# Autodesk Inventor assembly: Femto
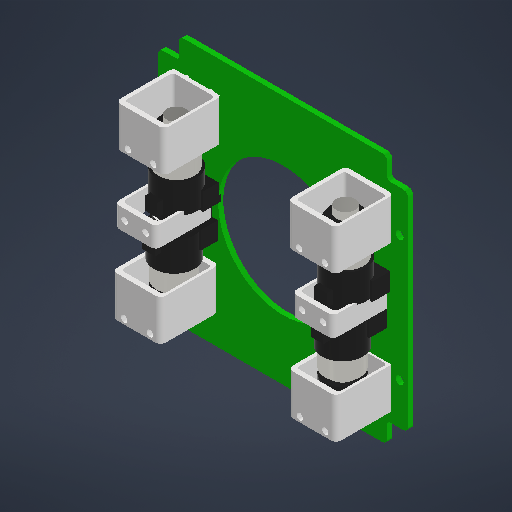
[picture p0: Inventor's stored thumbnail of the model, 512x512]
Saved by Autodesk Inventor 2026.1 (Build 301233020, 233B)
## iProperties
Created: 2025-11-06
Part Number: Femto
Document SubType Name: Assembly
Designer: SPEL
Author: SPEL
## Documents named in this file (5)
- C:\Users\patri\Desktop\SPEL\Femto\CAD\Femto.iam
- C:\Users\patri\Desktop\SPEL\Femto\CAD\PCB.ipt
- C:\Users\patri\Desktop\SPEL\Femto\CAD\injector femto.ipt
- C:\Users\patri\Desktop\SPEL\Femto\CAD\soporte inyector medio.ipt
- C:\Users\patri\Desktop\SPEL\Femto\CAD\soporte inyector salida.ipt
## Components (11 placed, 4 different names)
1. PCB:1
2. injector femto:1 — Coincidencia:5
3. injector femto:2 — Coincidencia:6
4. injector femto:3 — Coincidencia:6
5. injector femto:4 — Coincidencia:5
6. soporte inyector medio:1
7. soporte inyector salida:1
8. soporte inyector medio:2
9. soporte inyector salida:2
10. soporte inyector salida:3
11. soporte inyector salida:4
## Relationships (2: Mate 2)
- Coincidencia:5 [Mate]: injector femto:1 ↔ injector femto:4
- Coincidencia:6 [Mate]: injector femto:2 ↔ injector femto:3
